# Autodesk Inventor assembly: Assembly1
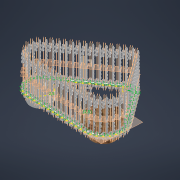
[picture p0: Inventor's stored thumbnail of the model, 180x180]
Saved by Autodesk Inventor 2022 (Build 260153000, 153)
## iProperties
Created: 2021-12-29
Part Number: Assembly1
Document SubType Name: Assembly
Designer: MatusBarany
Author: MatusBarany
## Documents named in this file (8)
- C:\Users\Public\Documents\Autodesk\Inventor 2022\Projects\wall-e\Assembly1.iam
- C:\Users\Public\Documents\Autodesk\Inventor 2022\Projects\wall-e\chain ink.ipt
- C:\Users\Public\Documents\Autodesk\Inventor 2022\Projects\wall-e\chain ink_outer.ipt
- C:\Users\Public\Documents\Autodesk\Inventor 2022\Projects\wall-e\male_koliesko.ipt
- C:\Users\Public\Documents\Autodesk\Inventor 2022\Projects\wall-e\velke_koleso.ipt
- C:\Users\Public\Documents\Autodesk\Inventor 2022\Projects\wall-e\stredne_koleso.ipt
- C:\Users\Public\Documents\Autodesk\Inventor 2022\Projects\wall-e\path of chain.ipt
- C:\Users\Public\Documents\Autodesk\Inventor 2022\Projects\wall-e\onePart_chain.ipt
## Components (57 placed, 7 different names)
1. chain ink:1 — Cylindrical:1, Cylindrical:4
2. chain ink_outer:1 — Cylindrical:1
3. chain ink_outer:2 — Cylindrical:4
4. male_koliesko:1
5. velke_koleso:1 — Flush:1
6. stredne_koleso:1
7. path of chain:1 — Mate:2, Mate:3
8. onePart_chain:1 — Mate:1, Mate:2, Mate:3
9. onePart_chain:2
10. onePart_chain:3
11. onePart_chain:4
12. onePart_chain:5
13. onePart_chain:6
14. onePart_chain:7
15. onePart_chain:8
16. onePart_chain:9
17. onePart_chain:10
18. onePart_chain:11
19. onePart_chain:12
20. onePart_chain:13
21. onePart_chain:14
22. onePart_chain:15
23. onePart_chain:16
24. onePart_chain:17
25. onePart_chain:18
26. onePart_chain:19
27. onePart_chain:20
28. onePart_chain:21
29. onePart_chain:22
30. onePart_chain:23
31. onePart_chain:24
32. onePart_chain:25
33. onePart_chain:26
34. onePart_chain:27
35. onePart_chain:28
36. onePart_chain:29
37. onePart_chain:30
38. onePart_chain:31
39. onePart_chain:32
40. onePart_chain:33
41. onePart_chain:34
42. onePart_chain:35
43. onePart_chain:36
44. onePart_chain:37
45. onePart_chain:38
46. onePart_chain:39
47. onePart_chain:40
48. onePart_chain:41
49. onePart_chain:42
50. onePart_chain:43
51. onePart_chain:44
52. onePart_chain:45
53. onePart_chain:46
54. onePart_chain:47
55. onePart_chain:48
56. onePart_chain:49
57. onePart_chain:50
## Component patterns: (50 elements, first: onePart_chain:1)
## Relationships (6: Mate 3, CylindricalJoint 2, Flush 1)
- Cylindrical:1: chain ink:1 ↔ chain ink_outer:1
- Cylindrical:4: chain ink:1 ↔ chain ink_outer:2
- Flush:1 (-1.5 mm): velke_koleso:1
- Mate:1: onePart_chain:1
- Mate:2: path of chain:1 ↔ onePart_chain:1
- Mate:3: path of chain:1 ↔ onePart_chain:1
